# Autodesk Inventor assembly: BasePlate
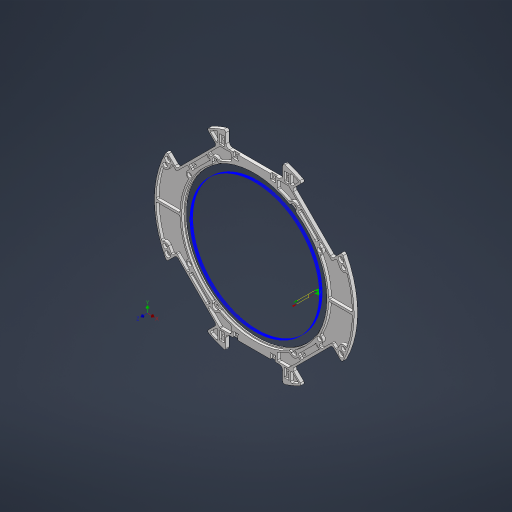
[picture p0: Inventor's stored thumbnail of the model, 512x512]
Saved by Autodesk Inventor 2024.2 (Build 282272000, 272)
## iProperties
Created: 2024-01-15
Part Number: BasePlate
Document SubType Name: Assembly
Designer: Hanaoka
Author: Hanaoka
## Documents named in this file (2)
- G:\共有ドライブ\reRo\05_個人\hanaoka\inventor\CAMpath\BasePlate.iam
- G:\共有ドライブ\reRo\05_個人\hanaoka\inventor\BasePlate.ipt
## Components (1 placed, 1 different names)
1. BasePlate:1 — メイト:1, メイト:2, 正接:1
## Relationships (3: Mate 2, Tangent 1)
- メイト:1 [Mate]: BasePlate:1
- メイト:2 [Mate] (14 mm): BasePlate:1
- 正接:1 [Tangent] (1 mm): BasePlate:1
